# Autodesk Inventor assembly: Leadscrew Constraint Front for 4040 - Assembly
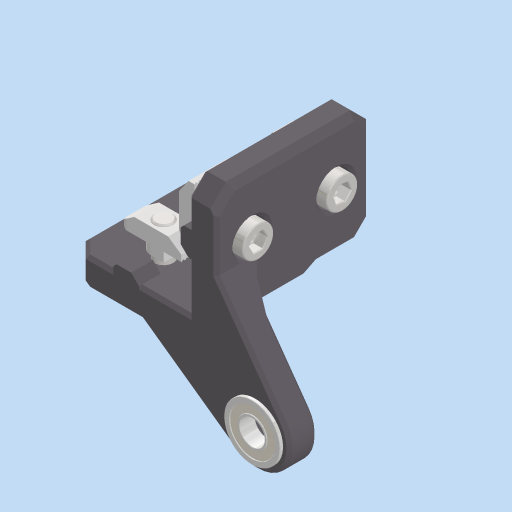
[picture p0: Inventor's stored thumbnail of the model, 512x512]
Saved by Autodesk Inventor 2023.2 (Build 272271000, 271)
## iProperties
Created: 2023-11-23
Part Number: Leadscrew Constraint Front for 4040 - Assembly
Document SubType Name: Assembly
Designer: Nils Bade
Author: Nils Bade
## Documents named in this file (6)
- C:\Users\nilsb\Documents\Inventor\Projektarbeit-Bade\RatRig_modified\Leadscrew Constraint Front for 4040 - Assembly.iam
- C:\Users\nilsb\Documents\Inventor\Projektarbeit-Bade\RatRig_modified\Leadscrew Constraint Front for 4040.ipt
- Leadscrew Constraint Front for 4040.ipt
- C:\Users\nilsb\Documents\Inventor\Projektarbeit-Bade\Schrauben\Cap Head Screw M6x16.ipt
- C:\Users\nilsb\Documents\Inventor\Projektarbeit-Bade\RatRig_modified\T-NUT - DropIn 4040 SERIES - M6.ipt
- C:\Users\nilsb\Documents\Inventor\Projektarbeit-Bade\RatRig_Standards\Ball Bearing - F688ZZ v1.ipt
## Components (10 placed, 4 different names)
1. Leadscrew Constraint Front for 4040:1 — Passend:13, Passend:14, Passend:15, Passend:16, Winkel:1, Winkel:2, Winkel:3, Winkel:4, Passend:17, Passend:18, Passend:19, Passend:20, Passend:21, Passend:22, Passend:23, Passend:24, Passend:25, Passend:26, Passend:27, Passend:28, Passend:29, Passend:30
2. Cap Head Screw M6x16:1 — Passend:19, Passend:27
3. Cap Head Screw M6x16:2 — Passend:24, Passend:28
4. Cap Head Screw M6x16:3 — Passend:26, Passend:30
5. Cap Head Screw M6x16:4 — Passend:25, Passend:29
6. T-NUT - DROP IN TYPE FOR 40 SERIES - M6:1 — Passend:15, Winkel:2, Passend:20
7. T-NUT - DROP IN TYPE FOR 40 SERIES - M6:2 — Passend:14, Winkel:4, Passend:23
8. T-NUT - DROP IN TYPE FOR 40 SERIES - M6:3 — Passend:16, Winkel:1, Passend:21
9. T-NUT - DROP IN TYPE FOR 40 SERIES - M6:4 — Passend:13, Winkel:3, Passend:22
10. Ball Bearing - F688ZZ v1:1 — Passend:17, Passend:18
## Relationships (22: Mate 18, Angle 4)
- Passend:13 [Mate] (5.5 mm): Leadscrew Constraint Front for 4040:1 ↔ T-NUT - DROP IN TYPE FOR 40 SERIES - M6:4
- Passend:14 [Mate] (5.5 mm): Leadscrew Constraint Front for 4040:1 ↔ T-NUT - DROP IN TYPE FOR 40 SERIES - M6:2
- Passend:15 [Mate] (5.5 mm): Leadscrew Constraint Front for 4040:1 ↔ T-NUT - DROP IN TYPE FOR 40 SERIES - M6:1
- Passend:16 [Mate] (5.5 mm): Leadscrew Constraint Front for 4040:1 ↔ T-NUT - DROP IN TYPE FOR 40 SERIES - M6:3
- Winkel:1 [Angle] (0 deg): Leadscrew Constraint Front for 4040:1 ↔ T-NUT - DROP IN TYPE FOR 40 SERIES - M6:3
- Winkel:2 [Angle] (0 deg): Leadscrew Constraint Front for 4040:1 ↔ T-NUT - DROP IN TYPE FOR 40 SERIES - M6:1
- Winkel:3 [Angle] (0 deg): Leadscrew Constraint Front for 4040:1 ↔ T-NUT - DROP IN TYPE FOR 40 SERIES - M6:4
- Winkel:4 [Angle] (0 deg): Leadscrew Constraint Front for 4040:1 ↔ T-NUT - DROP IN TYPE FOR 40 SERIES - M6:2
- Passend:17 [Mate]: Leadscrew Constraint Front for 4040:1 ↔ Ball Bearing - F688ZZ v1:1
- Passend:18 [Mate]: Leadscrew Constraint Front for 4040:1 ↔ Ball Bearing - F688ZZ v1:1
- Passend:19 [Mate]: Leadscrew Constraint Front for 4040:1 ↔ Cap Head Screw M6x16:1
- Passend:20 [Mate]: Leadscrew Constraint Front for 4040:1 ↔ T-NUT - DROP IN TYPE FOR 40 SERIES - M6:1
- Passend:21 [Mate]: Leadscrew Constraint Front for 4040:1 ↔ T-NUT - DROP IN TYPE FOR 40 SERIES - M6:3
- Passend:22 [Mate]: Leadscrew Constraint Front for 4040:1 ↔ T-NUT - DROP IN TYPE FOR 40 SERIES - M6:4
- Passend:23 [Mate]: Leadscrew Constraint Front for 4040:1 ↔ T-NUT - DROP IN TYPE FOR 40 SERIES - M6:2
- Passend:24 [Mate]: Leadscrew Constraint Front for 4040:1 ↔ Cap Head Screw M6x16:2
- Passend:25 [Mate]: Leadscrew Constraint Front for 4040:1 ↔ Cap Head Screw M6x16:4
- Passend:26 [Mate]: Leadscrew Constraint Front for 4040:1 ↔ Cap Head Screw M6x16:3
- Passend:27 [Mate]: Leadscrew Constraint Front for 4040:1 ↔ Cap Head Screw M6x16:1
- Passend:28 [Mate]: Leadscrew Constraint Front for 4040:1 ↔ Cap Head Screw M6x16:2
- Passend:29 [Mate]: Leadscrew Constraint Front for 4040:1 ↔ Cap Head Screw M6x16:4
- Passend:30 [Mate]: Leadscrew Constraint Front for 4040:1 ↔ Cap Head Screw M6x16:3
